# Autodesk Inventor assembly: B3M-SC-1040-A_with_ClampHorn_AND_FreeHorn
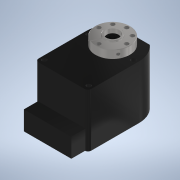
[picture p0: Inventor's stored thumbnail of the model, 180x180]
Saved by Autodesk Inventor 2022.3 (Build 263350000, 350)
## iProperties
Created: 2022-03-18
Part Number: B3M-SC-1040-A_with_ClampHorn_AND_FreeHorn
Document SubType Name: Assembly
Designer: MasatoKubotera
Author: MasatoKubotera
## Documents named in this file (4)
- C:\Users\Masato\Desktop\SUSTAINA-OP\ReadyMade\KONDO\B3M-SC-1040-A_with_ClampHorn_AND_FreeHorn.iam
- C:\Users\Masato\Desktop\SUSTAINA-OP\ReadyMade\KONDO\B3M-SC-1040-A_with_ClampHorn.iam
- C:\Users\Masato\Desktop\SUSTAINA-OP\ReadyMade\KONDO\FreeHorn.ipt
- C:\Users\Masato\Desktop\SUSTAINA-OP\ReadyMade\KONDO\FreeHorn_Screw.ipt
## Components (3 placed, 3 different names)
1. B3M-SC-1040-A_with_ClampHorn:1 [sub-assembly] — メイト:1, メイト:2, メイト:3, 挿入:1, 挿入:2
2. FreeHorn_:1 — 挿入:1
3. FreeHorn_Screw:1 — 挿入:2
## Relationships (5: Mate 3, Insert 2)
- メイト:1 [Mate]: B3M-SC-1040-A_with_ClampHorn:1
- メイト:2 [Mate]: B3M-SC-1040-A_with_ClampHorn:1
- メイト:3 [Mate]: B3M-SC-1040-A_with_ClampHorn:1
- 挿入:1 [Insert]: B3M-SC-1040-A_with_ClampHorn:1 ↔ FreeHorn_:1
- 挿入:2 [Insert]: B3M-SC-1040-A_with_ClampHorn:1 ↔ FreeHorn_Screw:1
